# Autodesk Inventor assembly: assembly_support
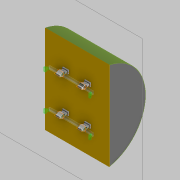
[picture p0: Inventor's stored thumbnail of the model, 180x180]
Saved by Autodesk Inventor 2021 (Build 250183000, 183)
## iProperties
Created: 2021-05-11
Part Number: assembly_support
Document SubType Name: Assembly
Designer: Watchdog
Author: Watchdog
## Documents named in this file (7)
- C:\Users\Watchdog\OneDrive - Flinders\Advn Mech Design Shared\6_Development\2_Design\inventor\support\assembly_support.iam
- C:\Users\Watchdog\OneDrive - Flinders\Advn Mech Design Shared\6_Development\2_Design\inventor\support\support_weldAssembly.iam
- C:\Users\Watchdog\OneDrive - Flinders\Advn Mech Design Shared\6_Development\2_Design\inventor\support\support_sandwichPlate.ipt
- C:\Users\Watchdog\OneDrive - Flinders\Advn Mech Design Shared\6_Development\2_Design\inventor\support\roof_bar\ext_roof bar assembly.iam
- C:\Users\Watchdog\OneDrive - Flinders\Advn Mech Design Shared\6_Development\2_Design\inventor\connection\assembly_connector.iam
- C:\Users\Watchdog\OneDrive - Flinders\Advn Mech Design Shared\6_Development\2_Design\inventor\support\support_frameAssembly.iam
- C:\Users\Watchdog\OneDrive - Flinders\Advn Mech Design Shared\6_Development\2_Design\inventor\cover\cover.iam
## Components (11 placed, 6 different names)
1. support_weldAssembly:1 [sub-assembly] — Flush:1, Mate:6, Mate:7
2. support_weldAssembly:2 [sub-assembly] — Mate:5, Flush:2, Mate:8, Mate:25
3. support_sandwichPlate:1 — Flush:1, Mate:5, Flush:2, Mate:6, Mate:7, Mate:8
4. ext_roof bar assembly:1 [sub-assembly] — Flush:6, Flush:7, Flush:8, Mate:15, Mate:16, Mate:18, Mate:20
5. ext_roof bar assembly:2 [sub-assembly] — Flush:3, Flush:4, Flush:5, Flush:6, Flush:7, Flush:8, Flush:9, Mate:11, Mate:13, Mate:14
6. assembly_connector:1 [sub-assembly] — Mate:9, Flush:9, Mate:10, Mate:11
7. support_frameAssembly:1 [sub-assembly] — Mate:22, Mate:23, Mate:24
8. cover:1 [sub-assembly] — Mate:9, Mate:10, Mate:12, Mate:17, Mate:19, Mate:21, Mate:22, Mate:23, Mate:24, Mate:25
9. assembly_connector:2 [sub-assembly] — Mate:12, Mate:13, Mate:14
10. assembly_connector:3 [sub-assembly] — Mate:15, Mate:16, Mate:17
11. assembly_connector:4 [sub-assembly] — Mate:18, Mate:19, Mate:20
## Relationships (30: Mate 21, Flush 9)
- Flush:1: support_weldAssembly:1 ↔ support_sandwichPlate:1
- Mate:5: support_weldAssembly:2 ↔ support_sandwichPlate:1
- Flush:2: support_weldAssembly:2 ↔ support_sandwichPlate:1
- Mate:6: support_weldAssembly:1 ↔ support_sandwichPlate:1
- Mate:7: support_weldAssembly:1 ↔ support_sandwichPlate:1
- Mate:8: support_weldAssembly:2 ↔ support_sandwichPlate:1
- Flush:3: ext_roof bar assembly:2
- Flush:4: ext_roof bar assembly:2
- Flush:5: ext_roof bar assembly:2
- Flush:6 (900 mm): ext_roof bar assembly:1 ↔ ext_roof bar assembly:2
- Flush:7: ext_roof bar assembly:1 ↔ ext_roof bar assembly:2
- Flush:8: ext_roof bar assembly:1 ↔ ext_roof bar assembly:2
- Mate:9: assembly_connector:1 ↔ cover:1
- Flush:9: ext_roof bar assembly:2 ↔ assembly_connector:1
- Mate:10: assembly_connector:1 ↔ cover:1
- Mate:11: ext_roof bar assembly:2 ↔ assembly_connector:1
- Mate:12: cover:1 ↔ assembly_connector:2
- Mate:13: ext_roof bar assembly:2 ↔ assembly_connector:2
- Mate:14: ext_roof bar assembly:2 ↔ assembly_connector:2
- Mate:15: ext_roof bar assembly:1 ↔ assembly_connector:3
- Mate:16: ext_roof bar assembly:1 ↔ assembly_connector:3
- Mate:17: cover:1 ↔ assembly_connector:3
- Mate:18: ext_roof bar assembly:1 ↔ assembly_connector:4
- Mate:19: cover:1 ↔ assembly_connector:4
- Mate:20: ext_roof bar assembly:1 ↔ assembly_connector:4
- Mate:21: cover:1
- Mate:22: support_frameAssembly:1 ↔ cover:1
- Mate:23: support_frameAssembly:1 ↔ cover:1
- Mate:24: support_frameAssembly:1 ↔ cover:1
- Mate:25: support_weldAssembly:2 ↔ cover:1
